# Autodesk Inventor assembly: Dropdown_Assembly_V3
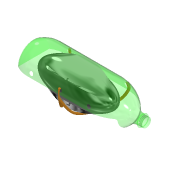
[picture p0: Inventor's stored thumbnail of the model, 180x180]
Saved by Autodesk Inventor 2021 (Build 250183000, 183)
## iProperties
Created: 2020-07-20
Part Number: Dropdown_Assembly_V3
Document SubType Name: Assembly
Designer: cameron
Author: cameron
## Documents named in this file (4)
- C:\Users\camer\Git\Sure2020-DropdownSystem\InventorDropsonde\Dropdown_Assembly_V3.iam
- C:\Users\camer\Git\Sure2020-DropdownSystem\InventorDropsonde\bottle_Half_V3.ipt
- C:\Users\camer\Git\Sure2020-DropdownSystem\InventorDropsonde\Dropsonde_V3.ipt
- C:\Users\camer\Git\Sure2020-DropdownSystem\InventorDropsonde\Drop_Rope.ipt
## Components (3 placed, 3 different names)
1. bottle_Half_V3:1 — Mate:1, Flush:1, Flush:2, Flush:3
2. Dropsonde_V3:1 — Mate:1
3. Drop_Rope:1 — Flush:1, Flush:2, Flush:3
## Relationships (4: Flush 3, Mate 1)
- Mate:1: bottle_Half_V3:1 ↔ Dropsonde_V3:1
- Flush:1: bottle_Half_V3:1 ↔ Drop_Rope:1
- Flush:2 (-167.869 mm): bottle_Half_V3:1 ↔ Drop_Rope:1
- Flush:3 (-122.5 mm): bottle_Half_V3:1 ↔ Drop_Rope:1
